# Autodesk Inventor assembly: Team5_assembly
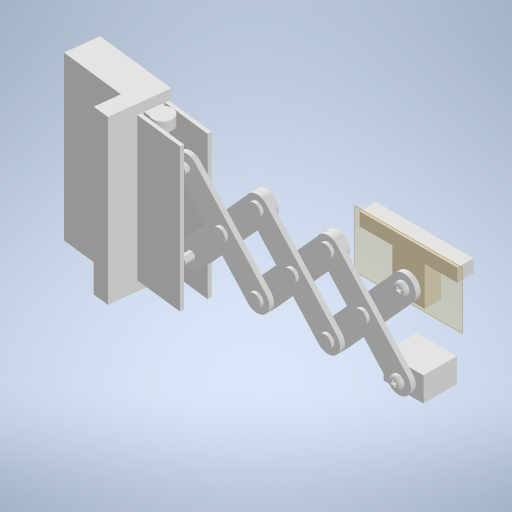
[picture p0: Inventor's stored thumbnail of the model, 512x512]
Saved by Autodesk Inventor 2024 (Build 280153000, 153)
## iProperties
Created: 2024-02-28
Part Number: Team5_assembly
Document SubType Name: Assembly
Designer: clbri
Author: clbri
## Documents named in this file (11)
- C:\Users\clbri\Downloads\Team5_assembly.iam
- C:\Users\clbri\Downloads\saanvi\top_bracket.ipt
- C:\Users\clbri\Downloads\Team5_screw.ipt
- C:\Users\clbri\Downloads\saanvi\DP3_linkage_extruded.ipt
- C:\Users\clbri\Downloads\saanvi\bracket_bottom1.ipt
- C:\Users\clbri\Downloads\saanvi\linkage_bolt_nut.ipt
- C:\Users\clbri\Downloads\saanvi\link_nut_bolt_end.ipt
- C:\Users\clbri\Downloads\saanvi\link_end_fixation.ipt
- C:\Users\clbri\Downloads\saanvi\guide_rod.ipt
- C:\Users\clbri\Downloads\saanvi\rod_end_fixation.ipt
- C:\Users\clbri\Downloads\guided hand 2.ipt
## Components (32 placed, 10 different names)
1. top_bracket:1 — Mate:1, Mate:2, Mate:4, Flush:1, Mate:75
2. Team5_screw:1 — Mate:1, Mate:2, Mate:5
3. DP3_linkage_extruded:1 — Mate:4, Mate:5, Mate:10, Mate:13, Mate:15, Mate:17, Mate:62, Mate:63
4. bracket_bottom1:1 — Mate:6, Mate:7, Flush:1
5. DP3_linkage_extruded:2 — Mate:14, Mate:16, Mate:18, Mate:20, Mate:55, Mate:56, Mate:57
6. DP3_linkage_extruded:3 — Mate:19, Mate:21, Mate:23, Mate:24, Mate:41, Mate:58, Mate:59, Mate:61
7. DP3_linkage_extruded:4 — Mate:15, Mate:16, Mate:17, Mate:18, Mate:19, Mate:22, Mate:23, Mate:25, Mate:28, Mate:33, Mate:34, Mate:37
8. DP3_linkage_extruded:5 — Mate:6, Mate:7, Mate:10, Mate:11, Mate:12, Mate:14, Mate:30, Mate:32, Mate:38, Mate:39
9. link_nut_bolt_end:1 — Mate:48, Mate:56
10. link_nut_bolt_end:2 — Mate:46, Mate:63
11. link_nut_bolt_end:3 — Mate:47, Mate:62
12. linkage_bolt_nut:4 — Mate:11, Mate:12, Mate:13, Mate:46
13. DP3_linkage_extruded:6 — Mate:20, Mate:21, Mate:24, Mate:27, Mate:31, Mate:35, Mate:36, Mate:40, Mate:44, Mate:60
14. linkage_bolt_nut:5 — Mate:22, Mate:25, Mate:54
15. linkage_bolt_nut:6 — Mate:30, Mate:32, Mate:49
16. linkage_bolt_nut:10 — Mate:28, Mate:34, Mate:47
17. linkage_bolt_nut:11 — Mate:31, Mate:35, Mate:50
18. linkage_bolt_nut:12 — Mate:33, Mate:37, Mate:48
19. linkage_bolt_nut:14 — Mate:27, Mate:36, Mate:53
20. Team5_screw:2 — Mate:38, Mate:39
21. link_end_fixation:1 — Mate:40, Mate:42, Mate:44, Mate:52, Mate:72
22. link_end_fixation:2 — Mate:41, Mate:43, Mate:51, Mate:73
23. guide_rod:1 — Mate:42, Mate:43, Mate:64, Mate:65, Mate:66, Mate:67
24. link_nut_bolt_end:4 — Mate:50, Mate:59
25. link_nut_bolt_end:5 — Mate:49, Mate:55
26. link_nut_bolt_end:6 — Mate:51, Mate:61
27. link_nut_bolt_end:7 — Mate:52, Mate:60
28. link_nut_bolt_end:8 — Mate:53, Mate:57
29. link_nut_bolt_end:9 — Mate:54, Mate:58
30. rod_end_fixation:1 — Mate:64, Mate:67, Mate:70, Mate:73
31. rod_end_fixation:2 — Mate:65, Mate:66, Mate:68, Mate:69, Mate:71, Mate:72
32. guided hand 2:1 — Mate:68, Mate:69, Mate:70, Mate:71, Mate:75
## Relationships (69: Mate 68, Flush 1)
- Mate:1: top_bracket:1 ↔ Team5_screw:1
- Mate:2 (3 mm): top_bracket:1 ↔ Team5_screw:1
- Mate:4: top_bracket:1 ↔ DP3_linkage_extruded:1
- Mate:5: Team5_screw:1 ↔ DP3_linkage_extruded:1
- Mate:6: bracket_bottom1:1 ↔ DP3_linkage_extruded:5
- Mate:7: bracket_bottom1:1 ↔ DP3_linkage_extruded:5
- Mate:10: DP3_linkage_extruded:1 ↔ DP3_linkage_extruded:5
- Mate:11: DP3_linkage_extruded:5 ↔ linkage_bolt_nut:4
- Mate:12: DP3_linkage_extruded:5 ↔ linkage_bolt_nut:4
- Mate:13: DP3_linkage_extruded:1 ↔ linkage_bolt_nut:4
- Mate:14: DP3_linkage_extruded:2 ↔ DP3_linkage_extruded:5
- Mate:15: DP3_linkage_extruded:1 ↔ DP3_linkage_extruded:4
- Mate:16: DP3_linkage_extruded:2 ↔ DP3_linkage_extruded:4
- Mate:17: DP3_linkage_extruded:1 ↔ DP3_linkage_extruded:4
- Mate:18: DP3_linkage_extruded:2 ↔ DP3_linkage_extruded:4
- Mate:19: DP3_linkage_extruded:3 ↔ DP3_linkage_extruded:4
- Mate:20: DP3_linkage_extruded:2 ↔ DP3_linkage_extruded:6
- Mate:21: DP3_linkage_extruded:3 ↔ DP3_linkage_extruded:6
- Mate:22: DP3_linkage_extruded:4 ↔ linkage_bolt_nut:5
- Mate:23: DP3_linkage_extruded:3 ↔ DP3_linkage_extruded:4
- Mate:24: DP3_linkage_extruded:3 ↔ DP3_linkage_extruded:6
- Mate:25: DP3_linkage_extruded:4 ↔ linkage_bolt_nut:5
- Mate:27: DP3_linkage_extruded:6 ↔ linkage_bolt_nut:14
- Mate:28: DP3_linkage_extruded:4 ↔ linkage_bolt_nut:10
- Mate:30: DP3_linkage_extruded:5 ↔ linkage_bolt_nut:6
- Mate:31: DP3_linkage_extruded:6 ↔ linkage_bolt_nut:11
- Mate:32: DP3_linkage_extruded:5 ↔ linkage_bolt_nut:6
- Mate:33: DP3_linkage_extruded:4 ↔ linkage_bolt_nut:12
- Mate:34: DP3_linkage_extruded:4 ↔ linkage_bolt_nut:10
- Mate:35: DP3_linkage_extruded:6 ↔ linkage_bolt_nut:11
- Mate:36: DP3_linkage_extruded:6 ↔ linkage_bolt_nut:14
- Mate:37: DP3_linkage_extruded:4 ↔ linkage_bolt_nut:12
- Flush:1 (2.25 mm): top_bracket:1 ↔ bracket_bottom1:1
- Mate:38: DP3_linkage_extruded:5 ↔ Team5_screw:2
- Mate:39: DP3_linkage_extruded:5 ↔ Team5_screw:2
- Mate:40: DP3_linkage_extruded:6 ↔ link_end_fixation:1
- Mate:41: DP3_linkage_extruded:3 ↔ link_end_fixation:2
- Mate:42: link_end_fixation:1 ↔ guide_rod:1
- Mate:43: link_end_fixation:2 ↔ guide_rod:1
- Mate:44: DP3_linkage_extruded:6 ↔ link_end_fixation:1
- Mate:46: link_nut_bolt_end:2 ↔ linkage_bolt_nut:4
- Mate:47: link_nut_bolt_end:3 ↔ linkage_bolt_nut:10
- Mate:48: link_nut_bolt_end:1 ↔ linkage_bolt_nut:12
- Mate:49: linkage_bolt_nut:6 ↔ link_nut_bolt_end:5
- Mate:50: linkage_bolt_nut:11 ↔ link_nut_bolt_end:4
- Mate:51: link_end_fixation:2 ↔ link_nut_bolt_end:6
- Mate:52: link_end_fixation:1 ↔ link_nut_bolt_end:7
- Mate:53: linkage_bolt_nut:14 ↔ link_nut_bolt_end:8
- Mate:54: linkage_bolt_nut:5 ↔ link_nut_bolt_end:9
- Mate:55: DP3_linkage_extruded:2 ↔ link_nut_bolt_end:5
- Mate:56: DP3_linkage_extruded:2 ↔ link_nut_bolt_end:1
- Mate:57: DP3_linkage_extruded:2 ↔ link_nut_bolt_end:8
- Mate:58: DP3_linkage_extruded:3 ↔ link_nut_bolt_end:9
- Mate:59: DP3_linkage_extruded:3 ↔ link_nut_bolt_end:4
- Mate:60: DP3_linkage_extruded:6 ↔ link_nut_bolt_end:7
- Mate:61: DP3_linkage_extruded:3 ↔ link_nut_bolt_end:6
- Mate:62: DP3_linkage_extruded:1 ↔ link_nut_bolt_end:3
- Mate:63: DP3_linkage_extruded:1 ↔ link_nut_bolt_end:2
- Mate:64: guide_rod:1 ↔ rod_end_fixation:1
- Mate:65: guide_rod:1 ↔ rod_end_fixation:2
- Mate:66: guide_rod:1 ↔ rod_end_fixation:2
- Mate:67: guide_rod:1 ↔ rod_end_fixation:1
- Mate:68: rod_end_fixation:2 ↔ guided hand 2:1
- Mate:69: rod_end_fixation:2 ↔ guided hand 2:1
- Mate:70: rod_end_fixation:1 ↔ guided hand 2:1
- Mate:71 (-14 mm): rod_end_fixation:2 ↔ guided hand 2:1
- Mate:72 (20 mm): link_end_fixation:1 ↔ rod_end_fixation:2
- Mate:73 (20 mm): link_end_fixation:2 ↔ rod_end_fixation:1
- Mate:75: top_bracket:1 ↔ guided hand 2:1
